# Autodesk Inventor assembly: Z-Arms
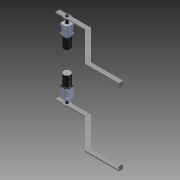
[picture p0: Inventor's stored thumbnail of the model, 180x180]
Saved by Autodesk Inventor 2013 (Build 170138000, 138)
## iProperties
Created: 2014-01-24
Part Number: Z-Arms
Document SubType Name: Assembly
Designer: Jarod
Author: Jarod
## Documents named in this file (4)
- D:\Robotics\FRC\2014\CAD\Robot\Pickup\Z-Arms.iam
- D:\Robotics\FRC\2014\CAD\Robot\Pickup\Z-PickupArm-L.ipt
- D:\Robotics\FRC\2014\CAD\Robot\Pickup\Z-PickupArm-R.ipt
- D:\Robotics\FRC\2014\CAD\Robot\Pickup\Imported Components\217-2 Stage Versaplanetary STEP\217-2 Stage Versaplanetary STEP.iam
## Components (4 placed, 3 different names)
1. Z-PickupArm-L:1 — Flush:1, Flush:2, Mate:3
2. Z-PickupArm-R:1 — Flush:1, Flush:2, Mate:2, Mate:4, Mate:5
3. 217-2 Stage Versaplanetary STEP:1 [sub-assembly] — Mate:2, Flush:3, Flush:4, Mate:4, Mate:5, Mate:6
4. 217-2 Stage Versaplanetary STEP:2 [sub-assembly] — Mate:3, Flush:3, Flush:4, Mate:6
## Relationships (9: Mate 5, Flush 4)
- Flush:1: Z-PickupArm-L:1 ↔ Z-PickupArm-R:1
- Flush:2: Z-PickupArm-L:1 ↔ Z-PickupArm-R:1
- Mate:2 (28.575 mm): Z-PickupArm-R:1 ↔ 217-2 Stage Versaplanetary STEP:1
- Mate:3 (28.575 mm): Z-PickupArm-L:1 ↔ 217-2 Stage Versaplanetary STEP:2
- Flush:3: 217-2 Stage Versaplanetary STEP:1 ↔ 217-2 Stage Versaplanetary STEP:2
- Flush:4: 217-2 Stage Versaplanetary STEP:1 ↔ 217-2 Stage Versaplanetary STEP:2
- Mate:4: Z-PickupArm-R:1 ↔ 217-2 Stage Versaplanetary STEP:1
- Mate:5: Z-PickupArm-R:1 ↔ 217-2 Stage Versaplanetary STEP:1
- Mate:6 (-387.35 mm): 217-2 Stage Versaplanetary STEP:1 ↔ 217-2 Stage Versaplanetary STEP:2
